# Autodesk Inventor assembly: 上半身
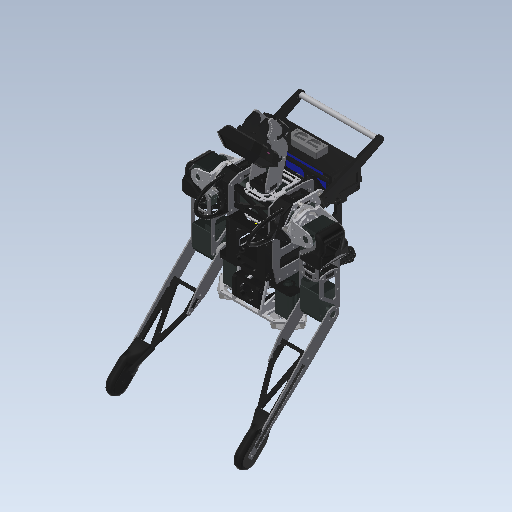
[picture p0: Inventor's stored thumbnail of the model, 512x512]
Saved by Autodesk Inventor 2020 (Build 240168000, 168)
## iProperties
Created: 2016-05-03
Part Number: 上半身
Document SubType Name: Assembly
Designer: hiroaki
Mass: 2583.03 g
Surface Area: 7335.68 cm^2
Volume: 1517.95 cm^3
Density: 1.70166 g/cm^3
Author: hiroaki
## Documents named in this file (7)
- C:\Users\naoki\Documents\Inventor\CitBrains\git_clone\OpenPlatform167\足首再設計1\OpenPlatform_ver3_0\上半身.iam
- C:\Users\naoki\Documents\Inventor\CitBrains\git_clone\OpenPlatform167\足首再設計1\OpenPlatform_ver3_0\上半身\胴体\胴体_1.iam
- C:\Users\naoki\Documents\Inventor\CitBrains\git_clone\OpenPlatform167\足首再設計1\OpenPlatform_ver3_0\上半身\腕\上腕_1.iam
- C:\Users\naoki\Documents\Inventor\CitBrains\git_clone\OpenPlatform167\足首再設計1\OpenPlatform_ver3_0\上半身\腕\前腕_1.iam
- C:\Users\naoki\Documents\Inventor\CitBrains\git_clone\OpenPlatform167\足首再設計1\OpenPlatform_ver3_0\上半身\腕\肩_1.iam
- C:\Users\naoki\Documents\Inventor\CitBrains\git_clone\OpenPlatform167\足首再設計1\OpenPlatform_ver3_0\上半身\頭\頭.iam
- C:\Users\naoki\Documents\Inventor\CitBrains\git_clone\OpenPlatform167\足首再設計1\OpenPlatform_ver3_0\上半身\腕\SideBumper.ipt
## Components (10 placed, 6 different names)
1. 胴体_1:1 [sub-assembly] — 挿入:5, 角度:1, 挿入:8, 角度:5, 角度:8, 角度:9, 挿入:10, 角度:10
2. 上腕_1:1 [sub-assembly] — 挿入:1, 挿入:3, 挿入:4, 角度:1, 角度:2, 角度:3, 角度:5, 角度:6, 角度:7, 角度:8, 角度:9, メイト:2, メイト:4, メイト:6
3. 前腕_1:1 [sub-assembly] — 挿入:1, 角度:3, 角度:4, 角度:6
4. 肩_1:1 [sub-assembly] — 挿入:3, 挿入:4, 挿入:5
5. 肩_1:2 [sub-assembly] — 挿入:7, 挿入:8
6. 上腕_1:2 [sub-assembly] — 挿入:7, 角度:2, 角度:7, 挿入:9, メイト:1, メイト:3, メイト:5
7. 前腕_1:2 [sub-assembly] — 角度:4, 挿入:9
8. 頭:1 [sub-assembly] — 挿入:10, 角度:10
9. SideBumper:1 — メイト:1, メイト:3, メイト:5
10. SideBumper:2 — メイト:2, メイト:4, メイト:6
## Relationships (24: Angle 10, Insert 8, Mate 6)
- 挿入:1 [Insert]: 上腕_1:1 ↔ 前腕_1:1
- 挿入:3 [Insert]: 上腕_1:1 ↔ 肩_1:1
- 挿入:4 [Insert]: 上腕_1:1 ↔ 肩_1:1
- 挿入:5 [Insert]: 胴体_1:1 ↔ 肩_1:1
- 角度:1 [Angle] (0 deg): 胴体_1:1 ↔ 上腕_1:1
- 挿入:7 [Insert]: 肩_1:2 ↔ 上腕_1:2
- 挿入:8 [Insert]: 胴体_1:1 ↔ 肩_1:2
- 角度:2 [Angle] (0 deg): 上腕_1:1 ↔ 上腕_1:2
- 角度:3 [Angle] (45 deg): 上腕_1:1 ↔ 前腕_1:1
- 角度:4 [Angle] (0 deg): 前腕_1:1 ↔ 前腕_1:2
- 角度:5 [Angle] (0 deg): 胴体_1:1 ↔ 上腕_1:1
- 角度:6 [Angle] (-90 deg): 上腕_1:1 ↔ 前腕_1:1
- 角度:7 [Angle] (0 deg): 上腕_1:1 ↔ 上腕_1:2
- 挿入:9 [Insert]: 上腕_1:2 ↔ 前腕_1:2
- 角度:8 [Angle] (0 deg): 胴体_1:1 ↔ 上腕_1:1
- 角度:9 [Angle] (0 deg): 胴体_1:1 ↔ 上腕_1:1
- 挿入:10 [Insert]: 胴体_1:1 ↔ 頭:1
- 角度:10 [Angle] (0 deg): 胴体_1:1 ↔ 頭:1
- メイト:1 [Mate]: 上腕_1:2 ↔ SideBumper:1
- メイト:2 [Mate]: 上腕_1:1 ↔ SideBumper:2
- メイト:3 [Mate]: 上腕_1:2 ↔ SideBumper:1
- メイト:4 [Mate]: 上腕_1:1 ↔ SideBumper:2
- メイト:5 [Mate]: 上腕_1:2 ↔ SideBumper:1
- メイト:6 [Mate]: 上腕_1:1 ↔ SideBumper:2
